# Autodesk Inventor assembly: 102.001.01_Vereinzelung_Gesamtbaugruppe
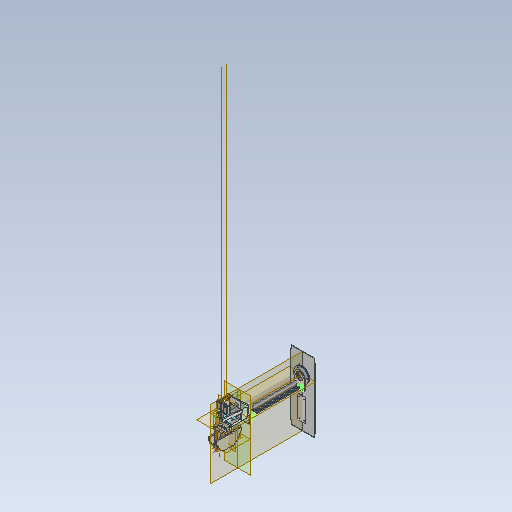
[picture p0: Inventor's stored thumbnail of the model, 512x512]
Saved by Autodesk Inventor 2021 (Build 250183000, 183)
## iProperties
Created: 2021-11-14
Part Number: 102.001.01_Vereinzelung_Gesamtbaugruppe
Document SubType Name: Assembly
Designer: Oliver Ungerer
Sending System: Creo  TM  4.0
KODE_ZEICHNUNGSNUMMER: TFVEM_100M
BENENNUNG: Vereinzelungsmechanismus
BEARBEITER_NAME: Ungerer O.
MASSE: 6.946813
PDMREV: 0.0+
PDMRL: Entwicklung
PROI_REVISION: 0
PROI_VERSION: 0+
PROI_RELEASE: Entwicklung
PTC_MODIFIED: True
PROI_CREATED_BY: Kantioler_adm
PROI_CREATED_ON: 07.03.2008 12:11:19
PROI_LOCATION: Root-Ordner/Pro_stds/Start_Files
MATERIALART: -
EINHEIT: ST
HERSTELLER_PREIS: 0.0
PRUEFER_NAME: Uo
PTC_ORGANIZATION_ID: Durst
PTC_WM_REVISION: 0
PTC_WM_ITERATION: 0
PTC_WM_VERSION: 0.0
PTC_WM_LIFECYCLE_STATE: Entwicklung
PTC_WM_LIFECYCLE: 02 Durst
PTC_WM_CREATED_BY: Oliver Ungerer (oungerer: Durst)
PTC_WM_CREATED_ON: 01.08.21
PTC_WM_MODIFIED_BY: Oliver Ungerer (oungerer: Durst)
PTC_WM_MODIFIED_ON: 01.08.21
AEND_INDEX: 0
VERSION: 0
STATUS: 0.0
Author: Oliver Ungerer
## Documents named in this file (26)
- \\u262868-sub21.your-storagebox.de@SSL\DavWWWRoot\Master_Projekt_SS_2021\Projektdaten\50_Modul_Vereinzelung\55_Konstruktion\102_Vereinzelung\102.001.01_Vereinzelung_Gesamtbaugruppe.iam
- \\u262868-sub21.your-storagebox.de@SSL\DavWWWRoot\Master_Projekt_SS_2021\Projektdaten\50_Modul_Vereinzelung\55_Konstruktion\102_Vereinzelung\TFVEM_1000.ipt
- \\u262868-sub21.your-storagebox.de@SSL\DavWWWRoot\Master_Projekt_SS_2021\Projektdaten\50_Modul_Vereinzelung\55_Konstruktion\102_Vereinzelung\TFVEM_1001.ipt
- \\u262868-sub21.your-storagebox.de@SSL\DavWWWRoot\Master_Projekt_SS_2021\Projektdaten\50_Modul_Vereinzelung\55_Konstruktion\102_Vereinzelung\202.001.01_Schieberbetaetigung.iam
- \\u262868-sub21.your-storagebox.de@SSL\DavWWWRoot\Master_Projekt_SS_2021\Projektdaten\50_Modul_Vereinzelung\55_Konstruktion\102_Vereinzelung\TFVEM_1002.ipt
- \\u262868-sub21.your-storagebox.de@SSL\DavWWWRoot\Master_Projekt_SS_2021\Projektdaten\50_Modul_Vereinzelung\55_Konstruktion\102_Vereinzelung\TFVEM_1003.ipt
- \\u262868-sub21.your-storagebox.de@SSL\DavWWWRoot\Master_Projekt_SS_2021\Projektdaten\50_Modul_Vereinzelung\55_Konstruktion\102_Vereinzelung\0001_FLASCHE.ipt
- \\u262868-sub21.your-storagebox.de@SSL\DavWWWRoot\Master_Projekt_SS_2021\Projektdaten\50_Modul_Vereinzelung\55_Konstruktion\102_Vereinzelung\TFVEM_1007.ipt
- \\u262868-sub21.your-storagebox.de@SSL\DavWWWRoot\Master_Projekt_SS_2021\Projektdaten\50_Modul_Vereinzelung\55_Konstruktion\102_Vereinzelung\TFVEM_1010.ipt
- \\u262868-sub21.your-storagebox.de@SSL\DavWWWRoot\Master_Projekt_SS_2021\Projektdaten\50_Modul_Vereinzelung\55_Konstruktion\102_Vereinzelung\_BALLUFF_BIS_M-305-ANTENNE.ipt
- \\u262868-sub21.your-storagebox.de@SSL\DavWWWRoot\Master_Projekt_SS_2021\Projektdaten\50_Modul_Vereinzelung\55_Konstruktion\102_Vereinzelung\TFVEM_1011.ipt
- \\u262868-sub21.your-storagebox.de@SSL\DavWWWRoot\Master_Projekt_SS_2021\Projektdaten\50_Modul_Vereinzelung\55_Konstruktion\102_Vereinzelung\BALLUFF_BCS_M18BBN1-PSC80D-EP02.ipt
- \\u262868-sub21.your-storagebox.de@SSL\DavWWWRoot\Master_Projekt_SS_2021\Projektdaten\50_Modul_Vereinzelung\55_Konstruktion\102_Vereinzelung\TFVEM_1018.ipt
- \\u262868-sub21.your-storagebox.de@SSL\DavWWWRoot\Master_Projekt_SS_2021\Projektdaten\50_Modul_Vereinzelung\55_Konstruktion\102_Vereinzelung\TFVEM_1015.ipt
- \\u262868-sub21.your-storagebox.de@SSL\DavWWWRoot\Master_Projekt_SS_2021\Projektdaten\50_Modul_Vereinzelung\55_Konstruktion\102_Vereinzelung\TFVEM_1016.ipt
- \\u262868-sub21.your-storagebox.de@SSL\DavWWWRoot\Master_Projekt_SS_2021\Projektdaten\50_Modul_Vereinzelung\55_Konstruktion\102_Vereinzelung\TFVEM_1017.ipt
- \\u262868-sub21.your-storagebox.de@SSL\DavWWWRoot\Master_Projekt_SS_2021\Projektdaten\50_Modul_Vereinzelung\55_Konstruktion\102_Vereinzelung\TFVEM_1019.ipt
- \\u262868-sub21.your-storagebox.de@SSL\DavWWWRoot\Master_Projekt_SS_2021\Projektdaten\50_Modul_Vereinzelung\55_Konstruktion\102_Vereinzelung\TFVEM_1020.ipt
- \\u262868-sub21.your-storagebox.de@SSL\DavWWWRoot\Master_Projekt_SS_2021\Projektdaten\50_Modul_Vereinzelung\55_Konstruktion\102_Vereinzelung\TFVEM_1021.ipt
- \\u262868-sub21.your-storagebox.de@SSL\DavWWWRoot\Master_Projekt_SS_2021\Projektdaten\50_Modul_Vereinzelung\55_Konstruktion\102_Vereinzelung\TFVEM_1022.ipt
- \\u262868-sub21.your-storagebox.de@SSL\DavWWWRoot\Master_Projekt_SS_2021\Projektdaten\50_Modul_Vereinzelung\55_Konstruktion\102_Vereinzelung\TFVEM_1023.ipt
- \\u262868-sub21.your-storagebox.de@SSL\DavWWWRoot\Master_Projekt_SS_2021\Projektdaten\50_Modul_Vereinzelung\55_Konstruktion\102_Vereinzelung\TFVEM_1024.ipt
- \\u262868-sub21.your-storagebox.de@SSL\DavWWWRoot\Master_Projekt_SS_2021\Projektdaten\50_Modul_Vereinzelung\55_Konstruktion\102_Vereinzelung\TFVEM_1025.ipt
- \\u262868-sub21.your-storagebox.de@SSL\DavWWWRoot\Master_Projekt_SS_2021\Projektdaten\50_Modul_Vereinzelung\55_Konstruktion\102_Vereinzelung\102.001.02_Anbindung_Vereinzelung.ipt
- \\u262868-sub21.your-storagebox.de@SSL\DavWWWRoot\Master_Projekt_SS_2021\Projektdaten\50_Modul_Vereinzelung\55_Konstruktion\102_Vereinzelung\102.001.03_Justage_Vereinzelung.ipt
- \\u262868-sub21.your-storagebox.de@SSL\DavWWWRoot\Master_Projekt_SS_2021\Projektdaten\50_Modul_Vereinzelung\55_Konstruktion\102_Vereinzelung\102.003.01_Anbindung_Vereinzelung.ipt
## Components (32 placed, 23 different names)
1. TFVEM_1000
2. TFVEM_1001 — Passend:1, Passend:13, Fluchtend:1, Passend:14
3. 202.001.01_Schieberbetaetigung [sub-assembly] — Passend:1, Passend:2, Passend:3, Passend:4
4. TFVEM_1002
5. TFVEM_1003 — Passend:6, Passend:7, Passend:8, Passend:10, Passend:12
6. 0001_FLASCHE
7. 0001_FLASCHE:1
8. TFVEM_1007
9. TFVEM_1010 — Passend:2, Passend:3, Passend:4
10. _BALLUFF_BIS_M-305-ANTENNE
11. TFVEM_1011
12. TFVEM_1011:1
13. BALLUFF_BCS_M18BBN1-PSC80D-EP02
14. BALLUFF_BCS_M18BBN1-PSC80D-EP02:1
15. TFVEM_1018
16. TFVEM_1015
17. TFVEM_1015:1
18. TFVEM_1016
19. TFVEM_1017
20. TFVEM_1019
21. TFVEM_1019:1
22. TFVEM_1019:2
23. TFVEM_1020
24. TFVEM_1021
25. TFVEM_1022
26. TFVEM_1023
27. TFVEM_1024
28. TFVEM_1025
29. 102.001.02_Anbindung_Vereinzelung:1 — Passend:6, Passend:7, Passend:8, Passend:9, Passend:11
30. 102.001.02_Anbindung_Vereinzelung:2 — Passend:9, Passend:10
31. 102.001.02_Anbindung_Vereinzelung:3 — Passend:11, Passend:12
32. 102.001.02_Anbindung_Vereinzelung:4 — Passend:13, Fluchtend:1, Passend:14
## Relationships (14: Mate 13, Flush 1)
- Passend:1 [Mate]: TFVEM_1001 ↔ 202.001.01_Schieberbetaetigung
- Passend:2 [Mate]: 202.001.01_Schieberbetaetigung ↔ TFVEM_1010
- Passend:3 [Mate]: 202.001.01_Schieberbetaetigung ↔ TFVEM_1010
- Passend:4 [Mate]: 202.001.01_Schieberbetaetigung ↔ TFVEM_1010
- Passend:6 [Mate]: TFVEM_1003 ↔ 102.001.02_Anbindung_Vereinzelung:1
- Passend:7 [Mate]: TFVEM_1003 ↔ 102.001.02_Anbindung_Vereinzelung:1
- Passend:8 [Mate] (25 mm): TFVEM_1003 ↔ 102.001.02_Anbindung_Vereinzelung:1
- Passend:9 [Mate]: 102.001.02_Anbindung_Vereinzelung:1 ↔ 102.001.02_Anbindung_Vereinzelung:2
- Passend:10 [Mate]: TFVEM_1003 ↔ 102.001.02_Anbindung_Vereinzelung:2
- Passend:11 [Mate]: 102.001.02_Anbindung_Vereinzelung:1 ↔ 102.001.02_Anbindung_Vereinzelung:3
- Passend:12 [Mate]: TFVEM_1003 ↔ 102.001.02_Anbindung_Vereinzelung:3
- Passend:13 [Mate]: TFVEM_1001 ↔ 102.001.02_Anbindung_Vereinzelung:4
- Fluchtend:1 [Flush]: TFVEM_1001 ↔ 102.001.02_Anbindung_Vereinzelung:4
- Passend:14 [Mate]: TFVEM_1001 ↔ 102.001.02_Anbindung_Vereinzelung:4
